# Autodesk Inventor assembly: Slide_Plate_LFinish
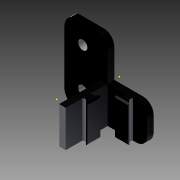
[picture p0: Inventor's stored thumbnail of the model, 180x180]
Saved by Autodesk Inventor 2014 (Build 180170000, 170)
## iProperties
Created: 2015-01-31
Part Number: Slide_Plate_LFinish
Document SubType Name: Assembly
Designer: Owner
Author: Owner
## Documents named in this file (3)
- C:\Users\Owner\Desktop\Lockdown Programs\Slide_Plate_LFinish.iam
- C:\Users\Owner\Desktop\Lockdown Programs\Slide_Plate_LTslot.ipt
- C:\Users\Owner\Desktop\Lockdown Programs\Slide_Plate_LExtResize.ipt
## Components (2 placed, 2 different names)
1. Slide_Plate_LExtResize:1 — Rigid:1
2. Slide_Plate_LTslot:1 — Rigid:1
## Relationships (1: WeldJoint 1)
- Rigid:1 [WeldJoint]: Slide_Plate_LExtResize:1 ↔ Slide_Plate_LTslot:1
